# Autodesk Inventor assembly: LF_2
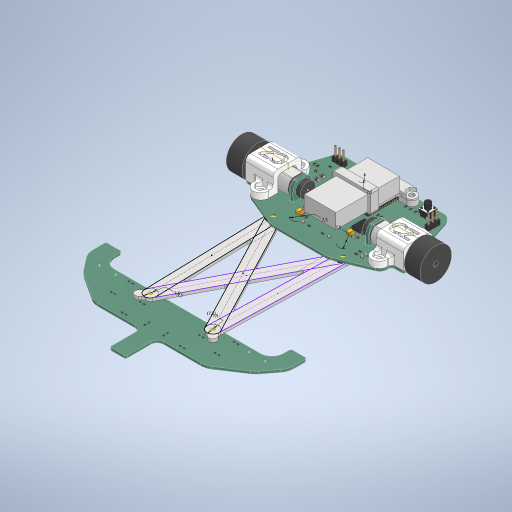
[picture p0: Inventor's stored thumbnail of the model, 512x512]
Saved by Autodesk Inventor 2023 (Build 270158000, 158)
## iProperties
Created: 2024-03-30
Part Number: LF_2
Document SubType Name: Assembly
Designer: Kamil
Author: Kamil
## Documents named in this file (11)
- C:\Users\kamil\Documents\PROJECTS - repos\Line_Follower_ZACZ\mechanics\LF_2.iam
- C:\Users\kamil\Documents\PROJECTS - repos\Line_Follower_ZACZ\mechanics\N20 Mini Micro Metall Gear Motor DC 3-6-12V v1.ipt
- C:\Users\kamil\Documents\PROJECTS - repos\Line_Follower_ZACZ\mechanics\kolko.ipt
- C:\Users\kamil\Documents\PROJECTS - repos\Line_Follower_ZACZ\mechanics\N20_Bracket_Extended_Pololu.ipt
- C:\Users\kamil\Documents\PROJECTS - repos\ModBot---Projekt-Zespolowy\mechanics\STEP\Płytka główna.ipt
- C:\Users\kamil\Documents\PROJECTS - repos\ModBot---Projekt-Zespolowy\mechanics\STEP\Płytka z czujnikami.ipt
- C:\Users\kamil\Documents\PROJECTS - repos\Line_Follower_ZACZ\mechanics\lacznik_2.ipt
- C:\Users\kamil\Documents\PROJECTS - repos\Line_Follower_ZACZ\mechanics\mocowanie.ipt
- C:\Users\kamil\Documents\PROJECTS - repos\Line_Follower_ZACZ\mechanics\li-pol_250.ipt
- C:\Users\kamil\Documents\PROJECTS - repos\Line_Follower_ZACZ\mechanics\trzymacz.ipt
- C:\Users\kamil\Documents\PROJECTS - repos\Line_Follower_ZACZ\mechanics\dol_trzymacz.ipt
## Components (15 placed, 10 different names)
1. N20 Mini Micro Metall Gear Motor DC 3-6-12V v1:1 — Zestawiające:27, Zestawiające:28, Zestawiające:29, Równoległe:1, Równoległe:2, Zestawiające:34, Równoległe:7, Zestawiające:40
2. N20 Mini Micro Metall Gear Motor DC 3-6-12V v1:2 — Zestawiające:30, Zestawiające:31, Zestawiające:32, Równoległe:3, Równoległe:4, Zestawiające:35, Równoległe:5, Zestawiające:37
3. kolko:1 — Zestawiające:30, Zestawiające:31
4. kolko:2 — Zestawiające:28, Zestawiające:29
5. N20_Bracket_Extended_Pololu:1 — Zestawiające:27, Równoległe:1, Równoległe:2
6. N20_Bracket_Extended_Pololu:2 — Zestawiające:32, Równoległe:3, Równoległe:4
7. Płytka główna:1 — Zestawiające:33, Zestawiające:34, Zestawiające:35, Zestawiające:36, Równoległe:6, Zestawiające:38, Zestawiające:39, Zestawiające:41, Zestawiające:42, Równoległe:8, Kątowe:1, Zestawiające:43, Równoległe:9, Zestawiające:44, Zestawiające:45, Zestawiające:47, Zestawiające:48, Równoległe:10, Równoległe:12, Zestawiające:49, Zestawiające:50, Zestawiające:51
8. N20_Bracket_Extended_Pololu:3 — Zestawiające:36, Równoległe:5, Zestawiające:37, Równoległe:6, Zestawiające:38
9. N20_Bracket_Extended_Pololu:4 — Zestawiające:39, Równoległe:7, Zestawiające:40, Zestawiające:41, Zestawiające:42
10. Płytka z czujnikami:1 — Kątowe:1, Zestawiające:43, Równoległe:9, Zestawiające:44, Zestawiające:46
11. lacznik_2:1 — Równoległe:8
12. mocowanie:1 — Zestawiające:45, Zestawiające:46, Zestawiające:47
13. li-pol_250:1 — Zestawiające:48, Równoległe:10, Równoległe:12
14. trzymacz:1 — Zestawiające:52, Zestawiające:53, Zestawiające:54
15. dol_trzymacz:1 — Zestawiające:49, Zestawiające:50, Zestawiające:51, Zestawiające:52, Zestawiające:53, Zestawiające:54
## Relationships (40: Mate 28, Flush 11, Angle 1)
- Zestawiające:27 [Mate]: N20 Mini Micro Metall Gear Motor DC 3-6-12V v1:1 ↔ N20_Bracket_Extended_Pololu:1
- Zestawiające:28 [Mate]: N20 Mini Micro Metall Gear Motor DC 3-6-12V v1:1 ↔ kolko:2
- Zestawiające:29 [Mate] (0.5 mm): N20 Mini Micro Metall Gear Motor DC 3-6-12V v1:1 ↔ kolko:2
- Równoległe:1 [Flush]: N20 Mini Micro Metall Gear Motor DC 3-6-12V v1:1 ↔ N20_Bracket_Extended_Pololu:1
- Równoległe:2 [Flush]: N20 Mini Micro Metall Gear Motor DC 3-6-12V v1:1 ↔ N20_Bracket_Extended_Pololu:1
- Zestawiające:30 [Mate] (0.5 mm): N20 Mini Micro Metall Gear Motor DC 3-6-12V v1:2 ↔ kolko:1
- Zestawiające:31 [Mate]: N20 Mini Micro Metall Gear Motor DC 3-6-12V v1:2 ↔ kolko:1
- Zestawiające:32 [Mate]: N20 Mini Micro Metall Gear Motor DC 3-6-12V v1:2 ↔ N20_Bracket_Extended_Pololu:2
- Równoległe:3 [Flush]: N20 Mini Micro Metall Gear Motor DC 3-6-12V v1:2 ↔ N20_Bracket_Extended_Pololu:2
- Równoległe:4 [Flush]: N20 Mini Micro Metall Gear Motor DC 3-6-12V v1:2 ↔ N20_Bracket_Extended_Pololu:2
- Zestawiające:33 [Mate]: Płytka główna:1
- Zestawiające:34 [Mate]: N20 Mini Micro Metall Gear Motor DC 3-6-12V v1:1 ↔ Płytka główna:1
- Zestawiające:35 [Mate]: N20 Mini Micro Metall Gear Motor DC 3-6-12V v1:2 ↔ Płytka główna:1
- Zestawiające:36 [Mate]: Płytka główna:1 ↔ N20_Bracket_Extended_Pololu:3
- Równoległe:5 [Flush]: N20 Mini Micro Metall Gear Motor DC 3-6-12V v1:2 ↔ N20_Bracket_Extended_Pololu:3
- Zestawiające:37 [Mate]: N20 Mini Micro Metall Gear Motor DC 3-6-12V v1:2 ↔ N20_Bracket_Extended_Pololu:3
- Równoległe:6 [Flush]: Płytka główna:1 ↔ N20_Bracket_Extended_Pololu:3
- Zestawiające:38 [Mate]: Płytka główna:1 ↔ N20_Bracket_Extended_Pololu:3
- Zestawiające:39 [Mate]: Płytka główna:1 ↔ N20_Bracket_Extended_Pololu:4
- Równoległe:7 [Flush]: N20 Mini Micro Metall Gear Motor DC 3-6-12V v1:1 ↔ N20_Bracket_Extended_Pololu:4
- Zestawiające:40 [Mate]: N20 Mini Micro Metall Gear Motor DC 3-6-12V v1:1 ↔ N20_Bracket_Extended_Pololu:4
- Zestawiające:41 [Mate]: Płytka główna:1 ↔ N20_Bracket_Extended_Pololu:4
- Zestawiające:42 [Mate]: Płytka główna:1 ↔ N20_Bracket_Extended_Pololu:4
- Równoległe:8 [Flush]: Płytka główna:1 ↔ lacznik_2:1
- Kątowe:1 [Angle] (0 deg): Płytka główna:1 ↔ Płytka z czujnikami:1
- Zestawiające:43 [Mate] (2 mm): Płytka główna:1 ↔ Płytka z czujnikami:1
- Równoległe:9 [Flush] (-13.525 mm): Płytka główna:1 ↔ Płytka z czujnikami:1
- Zestawiające:44 [Mate] (80 mm): Płytka główna:1 ↔ Płytka z czujnikami:1
- Zestawiające:45 [Mate]: Płytka główna:1 ↔ mocowanie:1
- Zestawiające:46 [Mate]: Płytka z czujnikami:1 ↔ mocowanie:1
- Zestawiające:47 [Mate]: Płytka główna:1 ↔ mocowanie:1
- Zestawiające:48 [Mate] (1 mm): Płytka główna:1 ↔ li-pol_250:1
- Równoległe:10 [Flush]: Płytka główna:1 ↔ li-pol_250:1
- Równoległe:12 [Flush] (-2.1 mm): Płytka główna:1 ↔ li-pol_250:1
- Zestawiające:49 [Mate]: Płytka główna:1 ↔ dol_trzymacz:1
- Zestawiające:50 [Mate]: Płytka główna:1 ↔ dol_trzymacz:1
- Zestawiające:51 [Mate]: Płytka główna:1 ↔ dol_trzymacz:1
- Zestawiające:52 [Mate]: trzymacz:1 ↔ dol_trzymacz:1
- Zestawiające:53 [Mate]: trzymacz:1 ↔ dol_trzymacz:1
- Zestawiające:54 [Mate]: trzymacz:1 ↔ dol_trzymacz:1
